# Autodesk Inventor assembly: _VK_Dreh-Station
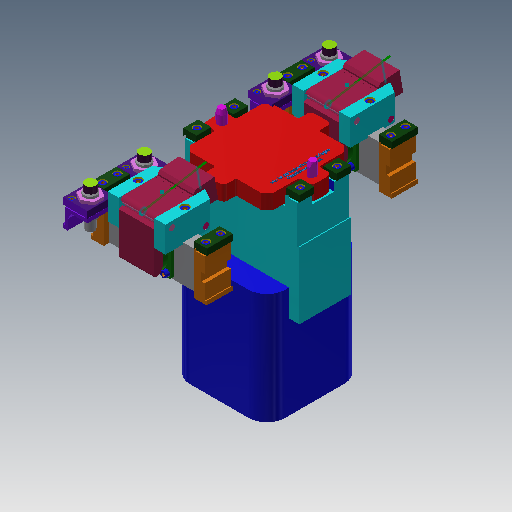
[picture p0: Inventor's stored thumbnail of the model, 512x512]
Saved by Autodesk Inventor 2019 (Build 230136000, 136)
## iProperties
Created: 2023-11-18
Part Number: _VK_Dreh-Station
Material: Generisch
Document SubType Name: Assembly
Designer: RP
Author: RP
## Documents named in this file (3)
- C:\Users\RP\Documents\Inventor\Projekt_Angelspule\_Verkettung\_VK_Hub-Dreh-Station.iam
- C:\Users\RP\Documents\Inventor\Projekt_Angelspule\_Verkettung\__VK_Stopper_Vor-Stopper_Einheit.iam
- C:\Users\RP\Documents\Inventor\Projekt_Angelspule\_Verkettung\__VK_Hub-Dreheinheit.iam
## Components (2 placed, 2 different names)
1. __VK_Stopper_Vor-Stopper_Einheit:1 [sub-assembly]
2. __VK_Hub-Dreheinheit:1 [sub-assembly] — Fluchtend:2, Fluchtend:5, Fluchtend:11
## Relationships (3: Flush 3)
- Fluchtend:2 [Flush]: __VK_Hub-Dreheinheit:1
- Fluchtend:5 [Flush]: __VK_Hub-Dreheinheit:1
- Fluchtend:11 [Flush]: __VK_Hub-Dreheinheit:1
